# Autodesk Inventor assembly: Waage
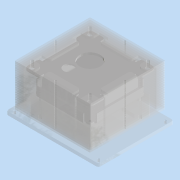
[picture p0: Inventor's stored thumbnail of the model, 180x180]
Saved by Autodesk Inventor 2022 (Build 260153000, 153)
## iProperties
Created: 2021-12-03
Part Number: Waage
Document SubType Name: Assembly
Designer: domin
Author: domin
## Documents named in this file (6)
- D:\Sync\Hivemind\1-MCI-Unterlagen\Master\Semester 3\Projekt 2\011_Kartesischer_Roboter_Modul\07-CAD Files\04-Waage\Waage.iam
- D:\Sync\Hivemind\1-MCI-Unterlagen\Master\Semester 3\Projekt 2\011_Kartesischer_Roboter_Modul\07-CAD Files\04-Waage\WaageBlechUnterseite.ipt
- D:\Sync\Hivemind\1-MCI-Unterlagen\Master\Semester 3\Projekt 2\011_Kartesischer_Roboter_Modul\07-CAD Files\04-Waage\WaageBlechOberseite.ipt
- D:\Sync\Hivemind\1-MCI-Unterlagen\Master\Semester 3\Projekt 2\011_Kartesischer_Roboter_Modul\07-CAD Files\04-Waage\WaagePlexiUnterseite.ipt
- D:\Sync\Hivemind\1-MCI-Unterlagen\Master\Semester 3\Projekt 2\011_Kartesischer_Roboter_Modul\07-CAD Files\04-Waage\WaagePlexi.iam
- D:\Sync\Hivemind\1-MCI-Unterlagen\Master\Semester 3\Projekt 2\011_Kartesischer_Roboter_Modul\07-CAD Files\04-Waage\WaagePlexiTurm.ipt
## Components (13 placed, 5 different names)
1. WaageBlechUnterseite:1 — Flush:1, Mate:1, Flush:2, Mate:2, Mate:3, Mate:4, Mate:5, Mate:6, Mate:7, Flush:3, Flush:4, Mate:11
2. WaageBlechOberseite:1 — Mate:2, Mate:3, Mate:4, Mate:8, Mate:9, Mate:10
3. WaagePlexiUnterseite:1 — Mate:5, Mate:6, Mate:7
4. WaagePlexi:1 [sub-assembly] — Mate:8, Mate:9, Mate:10
5. WaagePlexiTurm:1 — Flush:3, Flush:4, Mate:11
6. WaagePlexiTurm:2
7. WaagePlexiTurm:3
8. WaagePlexiTurm:4
9. WaagePlexiTurm:5
10. WaagePlexiTurm:6
11. WaagePlexiTurm:7
12. WaagePlexiTurm:8
13. WaagePlexiTurm:9
## Component patterns: (9 elements, first: WaagePlexiTurm:1)
## Relationships (15: Mate 11, Flush 4)
- Flush:1: WaageBlechUnterseite:1
- Mate:1: WaageBlechUnterseite:1
- Flush:2: WaageBlechUnterseite:1
- Mate:2 (-52.5 mm): WaageBlechUnterseite:1 ↔ WaageBlechOberseite:1
- Mate:3: WaageBlechUnterseite:1 ↔ WaageBlechOberseite:1
- Mate:4: WaageBlechUnterseite:1 ↔ WaageBlechOberseite:1
- Mate:5 (45 mm): WaageBlechUnterseite:1 ↔ WaagePlexiUnterseite:1
- Mate:6: WaageBlechUnterseite:1 ↔ WaagePlexiUnterseite:1
- Mate:7: WaageBlechUnterseite:1 ↔ WaagePlexiUnterseite:1
- Mate:8: WaageBlechOberseite:1 ↔ WaagePlexi:1
- Mate:9: WaageBlechOberseite:1 ↔ WaagePlexi:1
- Mate:10: WaageBlechOberseite:1 ↔ WaagePlexi:1
- Flush:3: WaageBlechUnterseite:1 ↔ WaagePlexiTurm:1
- Flush:4: WaageBlechUnterseite:1 ↔ WaagePlexiTurm:1
- Mate:11: WaageBlechUnterseite:1 ↔ WaagePlexiTurm:1
